# Autodesk Inventor assembly: Body
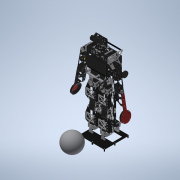
[picture p0: Inventor's stored thumbnail of the model, 180x180]
Saved by Autodesk Inventor 2020.4 (Build 244396000, 396)
## iProperties
Created: 2021-09-30
Part Number: Body
Document SubType Name: Assembly
Designer: Masato Kubotera
Mass: 3705.91 g
Surface Area: 12998.1 cm^2
Volume: 3273.31 cm^3
Density: 1.13216 g/cm^3
Author: Masato Kubotera
## Documents named in this file (4)
- C:\Users\Masato\Documents\Inventor\CIT Brains_Inventor\SUSTAINA-OP\Body.iam
- C:\Users\Masato\Documents\Inventor\CIT Brains_Inventor\SUSTAINA-OP\UpperBody\UpperBody.iam
- C:\Users\Masato\Documents\Inventor\CIT Brains_Inventor\SUSTAINA-OP\LowerBody\LowerBody.iam
- C:\Users\Masato\Documents\Inventor\CIT Brains_Inventor\SUSTAINA-OP\ReadyMade\Ball.ipt
## Components (4 placed, 3 different names)
1. UpperBody:1 [sub-assembly] — 挿入:1, フラッシュ:1, 挿入:2
2. LowerBody:1 [sub-assembly] — 挿入:1, フラッシュ:3, メイト:3, 角度:1
3. LowerBody:2 [sub-assembly] — 挿入:2, 角度:1
4. Ball:1 — 正接:1, メイト:1, メイト:2
## Relationships (9: Mate 3, Insert 2, Flush 2, Tangent 1, Angle 1)
- 正接:1 [Tangent]: Ball:1
- メイト:1 [Mate] (200 mm): Ball:1
- メイト:2 [Mate]: Ball:1
- 挿入:1 [Insert]: UpperBody:1 ↔ LowerBody:1
- フラッシュ:1 [Flush]: UpperBody:1
- フラッシュ:3 [Flush]: LowerBody:1
- メイト:3 [Mate]: LowerBody:1
- 挿入:2 [Insert]: UpperBody:1 ↔ LowerBody:2
- 角度:1 [Angle] (0 deg): LowerBody:1 ↔ LowerBody:2
